# Autodesk Inventor assembly: sub assembly 3
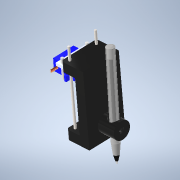
[picture p0: Inventor's stored thumbnail of the model, 180x180]
Saved by Autodesk Inventor 2021 (Build 250183000, 183)
## iProperties
Created: 2021-07-13
Part Number: sub assembly 3
Document SubType Name: Assembly
Designer: Michael Swaminathan
Author: Michael Swaminathan
## Documents named in this file (8)
- F:\Pattern Drawing Bot\Xy plotter Drawing Machine\sub assembly 3.iam
- F:\Pattern Drawing Bot\Xy plotter Drawing Machine\Guidance Rods.ipt
- F:\Pattern Drawing Bot\Xy plotter Drawing Machine\Pen Holder.ipt
- F:\Pattern Drawing Bot\Xy plotter Drawing Machine\Holding Stand.ipt
- F:\Pattern Drawing Bot\Xy plotter Drawing Machine\BIC Round Stic Pen Assembly.iam
- F:\Pattern Drawing Bot\Xy plotter Drawing Machine\Servo Motor Support.ipt
- F:\Pattern Drawing Bot\Xy plotter Drawing Machine\Servo motor support rods.ipt
- F:\Pattern Drawing Bot\Xy plotter Drawing Machine\Micro Servo SG90.ipt
## Components (9 placed, 7 different names)
1. Guidance Rods:1 — Insert:7
2. Guidance Rods:2 — Mate:6
3. Pen Holder:1 — Rigid:13, Insert:9
4. Holding Stand:1 — Mate:6, Insert:7, Insert:9
5. BIC Round Stic Pen Assembly:1 [sub-assembly] — Rigid:13
6. Servo Motor Support:1 — Rotational:10
7. Servo motor support rods:1 — Rotational:10
8. Servo motor support rods:2
9. Micro Servo SG90:1
## Relationships (5: Insert 2, Mate 1, WeldJoint 1, RevoluteJoint 1)
- Mate:6: Guidance Rods:2 ↔ Holding Stand:1
- Rigid:13 [WeldJoint] (19 mm): Pen Holder:1 ↔ BIC Round Stic Pen Assembly:1
- Insert:7 (13.5 mm): Guidance Rods:1 ↔ Holding Stand:1
- Rotational:10 [RevoluteJoint] (7.5 mm): Servo Motor Support:1 ↔ Servo motor support rods:1
- Insert:9 (-10 mm): Pen Holder:1 ↔ Holding Stand:1
